# Autodesk Inventor assembly: Boden_Ecke
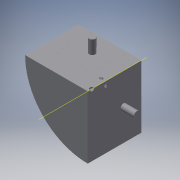
[picture p0: Inventor's stored thumbnail of the model, 180x180]
Saved by Autodesk Inventor 2019 (Build 230136000, 136)
## iProperties
Created: 2018-08-15
Part Number: Boden_Ecke
Document SubType Name: Assembly
Designer: Julia
Author: Julia
## Documents named in this file (3)
- C:\Users\Julia\Documents\Inventor\3D_Drucker_v01\Boden_Ecke.iam
- C:\Users\Julia\Documents\Inventor\3D_Drucker_v01\Einschub.ipt
- C:\Users\Julia\Documents\Inventor\3D_Drucker_v01\Ecke.ipt
## Components (3 placed, 2 different names)
1. Einschub:1 — Mate:2, Mate:4, Mate:5
2. Ecke:1 — Mate:1, Mate:2, Mate:3, Mate:4, Mate:5, Mate:6
3. Einschub:2 — Mate:1, Mate:3, Mate:6
## Relationships (6: Mate 6)
- Mate:1: Ecke:1 ↔ Einschub:2
- Mate:2: Einschub:1 ↔ Ecke:1
- Mate:3: Ecke:1 ↔ Einschub:2
- Mate:4: Einschub:1 ↔ Ecke:1
- Mate:5: Einschub:1 ↔ Ecke:1
- Mate:6: Ecke:1 ↔ Einschub:2
